# Autodesk Inventor assembly: 211-06
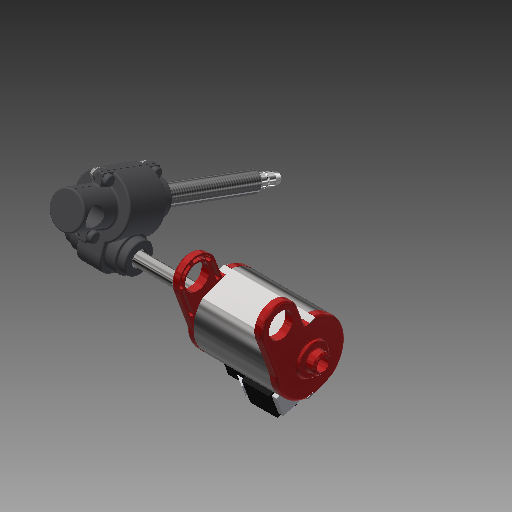
[picture p0: Inventor's stored thumbnail of the model, 512x512]
Saved by Autodesk Inventor 2019 (Build 230136000, 136)
## iProperties
Company: Autodesk Inc.
Created: 2008-01-21
Part Number: 211-06
Description: WORM DRIVE ASSEMBLY
Document SubType Name: Assembly
Designer: Autodesk Inc.
Mass: 260.873 g
Surface Area: 740.564 cm^2
Volume: 94.4535 cm^3
Density: 2.76193 g/cm^3
Author: Inventor
## Documents named in this file (4)
- C:\TEMP\Car Seat\Workspace\Front Worm Drive Assembly_MIR.iam
- C:\TEMP\Car Seat\Workspace\Front Drive Assembly_MIR.iam
- C:\TEMP\Car Seat\Workspace\Worm Drive Shaft.iam
- C:\TEMP\Car Seat\Workspace\Rear Ball Screw Shaft Assembly.iam
## Components (3 placed, 3 different names)
1. Rear Ball Screw Shaft Assembly:1 [sub-assembly] — Insert:1
2. Front Drive Assembly_MIR:1 [sub-assembly] — Insert:1, Mate:1, Insert:2, Mate:2
3. Worm Drive Shaft:1 [sub-assembly] — Mate:1, Insert:2
## Relationships (4: Insert 2, Mate 2)
- Insert:1: Rear Ball Screw Shaft Assembly:1 ↔ Front Drive Assembly_MIR:1
- Mate:1: Front Drive Assembly_MIR:1 ↔ Worm Drive Shaft:1
- Insert:2: Front Drive Assembly_MIR:1 ↔ Worm Drive Shaft:1
- Mate:2: Front Drive Assembly_MIR:1
